# Autodesk Inventor assembly: Canaleta 30x30 317mm
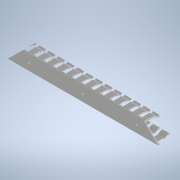
[picture p0: Inventor's stored thumbnail of the model, 180x180]
Saved by Autodesk Inventor 2021 (Build 250183000, 183)
## iProperties
Created: 2021-04-16
Part Number: Canaleta 30x30 317mm
Document SubType Name: Assembly
Designer: Nelson
Author: Nelson
## Documents named in this file (3)
- D:\Nelson\Documentos\Inventor\PAI_ElementosInternos\Canaleta 30x30 317mm.iam
- D:\Nelson\Documentos\Inventor\PAI_ElementosInternos\Cuerpo 30x30 317mm.ipt
- D:\Nelson\Documentos\Inventor\PAI_ElementosInternos\Tapa 30x30 317mm.ipt
## Components (2 placed, 2 different names)
1. Cuerpo 30x30 317mm:1 — Flush:1, Flush:2, Flush:3
2. Tapa 30x30 317mm:1 — Flush:1, Flush:2, Flush:3
## Relationships (3: Flush 3)
- Flush:1: Cuerpo 30x30 317mm:1 ↔ Tapa 30x30 317mm:1
- Flush:2: Cuerpo 30x30 317mm:1 ↔ Tapa 30x30 317mm:1
- Flush:3 (26 mm): Cuerpo 30x30 317mm:1 ↔ Tapa 30x30 317mm:1
